# Autodesk Inventor assembly: L_Unit_SR-W
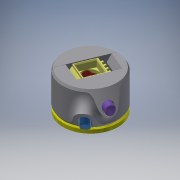
[picture p0: Inventor's stored thumbnail of the model, 180x180]
Saved by Autodesk Inventor 2018.3 (Build 223284000, 284)
## iProperties
Created: 2018-04-24
Part Number: L_Unit_SR-W
Material: 一般
Document SubType Name: Assembly
Designer: sktom
Author: sktom
## Documents named in this file (9)
- D:\CloudStrage\OneDrive\CADMech\HbSizeSMech\UnitWrist\L_Unit_SR-W.iam
- D:\CloudStrage\OneDrive\CADMech\HbSizeSMech\UnitWrist\Parts_SR-W\L_SR-W-01.ipt
- D:\CloudStrage\OneDrive\CADMech\HbSizeSMech\UnitWrist\Parts_SR-W\L_SR-W-02.ipt
- D:\CloudStrage\OneDrive\CADMech\HbSizeSMech\UnitWrist\Parts_SR-W\L_SR-W-03.ipt
- D:\CloudStrage\OneDrive\CADMech\HbSizeSMech\UnitWrist\Parts_SR-W\L_SR-W-04.ipt
- D:\CloudStrage\OneDrive\CADMech\HbSizeSMech\UnitWrist\Parts_SR-W\L_SR-W-05.ipt
- D:\CloudStrage\OneDrive\CADMech\HbSizeSMech\UnitWrist\Parts_SR-W\L_SR-W-06.ipt
- D:\CloudStrage\OneDrive\CADMech\HbSizeSMech\UnitWrist\Parts_SR-W\L_SR-W-07.ipt
- D:\CloudStrage\OneDrive\CADMech\HbSizeSMech\UnitWrist\Parts_SR-W\L_SR-W-08.ipt
## Components (8 placed, 8 different names)
1. L_SR-W-01:1 — リジッド:1
2. L_SR-W-03:1 — 挿入:6, 円柱状:1
3. L_SR-W-02:1 — 挿入:3, 挿入:5, 挿入:4, 挿入:6, メイト:1, リジッド:1, 円柱状:1, 円柱状:2
4. L_SR-W-04:1 — 挿入:2, 挿入:1, 挿入:3
5. L_SR-W-05:1 — 挿入:2, 挿入:1
6. L_SR-W-06:1 — リジッド:2
7. L_SR-W-07:1 — メイト:1, 円柱状:2, リジッド:2
8. L_SR-W-08:1 — 挿入:5, 挿入:4
## Relationships (11: Insert 6, WeldJoint 2, CylindricalJoint 2, Mate 1)
- 挿入:2 [Insert]: L_SR-W-04:1 ↔ L_SR-W-05:1
- 挿入:1 [Insert]: L_SR-W-04:1 ↔ L_SR-W-05:1
- 挿入:3 [Insert]: L_SR-W-02:1 ↔ L_SR-W-04:1
- 挿入:5 [Insert]: L_SR-W-02:1 ↔ L_SR-W-08:1
- 挿入:4 [Insert]: L_SR-W-02:1 ↔ L_SR-W-08:1
- 挿入:6 [Insert]: L_SR-W-03:1 ↔ L_SR-W-02:1
- メイト:1 [Mate] (0.5 mm): L_SR-W-02:1 ↔ L_SR-W-07:1
- リジッド:1 [WeldJoint]: L_SR-W-01:1 ↔ L_SR-W-02:1
- 円柱状:1 [CylindricalJoint]: L_SR-W-03:1 ↔ L_SR-W-02:1
- 円柱状:2 [CylindricalJoint]: L_SR-W-02:1 ↔ L_SR-W-07:1
- リジッド:2 [WeldJoint]: L_SR-W-06:1 ↔ L_SR-W-07:1
